# Autodesk Inventor assembly: 2SIDEROLLERASSEM
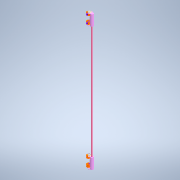
[picture p0: Inventor's stored thumbnail of the model, 180x180]
Saved by Autodesk Inventor 2022 (Build 260153000, 153)
## iProperties
Created: 2022-11-14
Part Number: 2SIDEROLLERASSEM
Document SubType Name: Assembly
Designer: matia
Author: matia
## Documents named in this file (3)
- C:\Users\matia\Desktop\1QuadMod\2SIDEROLLERASSEM.iam
- C:\Users\matia\Desktop\1QuadMod\blockrod.ipt
- C:\Users\matia\Desktop\1QuadMod\rollerassembly(v2).iam
## Components (3 placed, 2 different names)
1. blockrod:1 — Mate:1, Mate:2, Mate:3, Mate:4
2. rollerassembly(v2):1 [sub-assembly] — Mate:3, Mate:4
3. rollerassembly(v2):2 [sub-assembly] — Mate:1, Mate:2
## Relationships (4: Mate 4)
- Mate:1: blockrod:1 ↔ rollerassembly(v2):2
- Mate:2: blockrod:1 ↔ rollerassembly(v2):2
- Mate:3: blockrod:1 ↔ rollerassembly(v2):1
- Mate:4: blockrod:1 ↔ rollerassembly(v2):1
